# Autodesk Inventor assembly: Shoulder
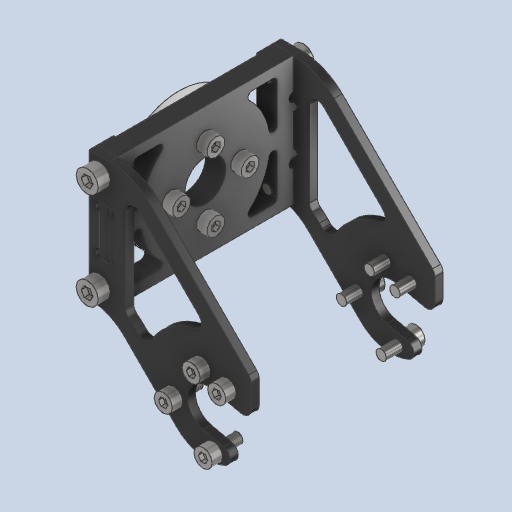
[picture p0: Inventor's stored thumbnail of the model, 512x512]
Saved by Autodesk Inventor 2022.3 (Build 263350000, 350)
## iProperties
Created: 2022-01-10
Part Number: Shoulder
Document SubType Name: Assembly
Designer: Masato Kubotera
Author: Masato Kubotera
## Documents named in this file (7)
- C:\Users\Masato\Documents\Inventor\CIT Brains\SUSTAINA-OP - mod\UpperBody\Arm\Shoulder.iam
- C:\Users\Masato\Documents\Inventor\CIT Brains\SUSTAINA-OP - mod\ReadyMade\Washer\TT-2532-20.ipt
- C:\Users\Masato\Documents\Inventor\CIT Brains\SUSTAINA-OP - mod\UpperBody\UpperBody_horn_frame.ipt
- C:\Users\Masato\Documents\Inventor\CIT Brains\SUSTAINA-OP - mod\UpperBody\Arm\Shoulder_side_frame.ipt
- C:\Users\Masato\Documents\Inventor\CIT Brains\SUSTAINA-OP - mod\ReadyMade\Screw\UC-2606.ipt
- C:\Users\Masato\Documents\Inventor\CIT Brains\SUSTAINA-OP - mod\ReadyMade\Screw\UC-0306.ipt
- C:\Users\Masato\Documents\Inventor\CIT Brains\SUSTAINA-OP - mod\ReadyMade\Screw\UC-2610.ipt
## Components (20 placed, 6 different names)
1. UpperBody_horn_frame:1 — メイト:1, メイト:2, メイト:3, 挿入:1, 挿入:2, 挿入:3, 挿入:4, 挿入:5, Insert:22, Insert:23, Insert:24, Insert:25
2. Shoulder_side_frame:1 — 挿入:2, 挿入:3, 挿入:6, 挿入:7, 挿入:8, 挿入:9, 挿入:18, 挿入:19
3. Shoulder_side_frame:2 — 挿入:4, 挿入:5, 挿入:10, 挿入:11, 挿入:12, 挿入:13, 挿入:20, 挿入:21
4. TT-2532-20:1 — 挿入:1
5. UC-2606:1 — 挿入:6
6. UC-2606:2 — 挿入:7
7. UC-2606:3 — 挿入:8
8. UC-2606:4 — 挿入:9
9. UC-2606:5 — 挿入:10
10. UC-2606:6 — 挿入:11
11. UC-2606:7 — 挿入:12
12. UC-2606:8 — 挿入:13
13. UC-0306:1 — 挿入:18
14. UC-0306:2 — 挿入:19
15. UC-0306:3 — 挿入:20
16. UC-0306:4 — 挿入:21
17. UC-2610:1 — Insert:23
18. UC-2610:2 — Insert:22
19. UC-2610:3 — Insert:25
20. UC-2610:4 — Insert:24
## Relationships (24: Insert 21, Mate 3)
- メイト:1 [Mate]: UpperBody_horn_frame:1
- メイト:2 [Mate]: UpperBody_horn_frame:1
- メイト:3 [Mate]: UpperBody_horn_frame:1
- 挿入:1 [Insert]: UpperBody_horn_frame:1 ↔ TT-2532-20:1
- 挿入:2 [Insert]: UpperBody_horn_frame:1 ↔ Shoulder_side_frame:1
- 挿入:3 [Insert]: UpperBody_horn_frame:1 ↔ Shoulder_side_frame:1
- 挿入:4 [Insert]: UpperBody_horn_frame:1 ↔ Shoulder_side_frame:2
- 挿入:5 [Insert]: UpperBody_horn_frame:1 ↔ Shoulder_side_frame:2
- 挿入:6 [Insert]: Shoulder_side_frame:1 ↔ UC-2606:1
- 挿入:7 [Insert]: Shoulder_side_frame:1 ↔ UC-2606:2
- 挿入:8 [Insert]: Shoulder_side_frame:1 ↔ UC-2606:3
- 挿入:9 [Insert]: Shoulder_side_frame:1 ↔ UC-2606:4
- 挿入:10 [Insert]: Shoulder_side_frame:2 ↔ UC-2606:5
- 挿入:11 [Insert]: Shoulder_side_frame:2 ↔ UC-2606:6
- 挿入:12 [Insert]: Shoulder_side_frame:2 ↔ UC-2606:7
- 挿入:13 [Insert]: Shoulder_side_frame:2 ↔ UC-2606:8
- 挿入:18 [Insert]: Shoulder_side_frame:1 ↔ UC-0306:1
- 挿入:19 [Insert]: Shoulder_side_frame:1 ↔ UC-0306:2
- 挿入:20 [Insert]: Shoulder_side_frame:2 ↔ UC-0306:3
- 挿入:21 [Insert]: Shoulder_side_frame:2 ↔ UC-0306:4
- Insert:22: UpperBody_horn_frame:1 ↔ UC-2610:2
- Insert:23: UpperBody_horn_frame:1 ↔ UC-2610:1
- Insert:24: UpperBody_horn_frame:1 ↔ UC-2610:4
- Insert:25: UpperBody_horn_frame:1 ↔ UC-2610:3
